# Autodesk Inventor assembly: blocoRolamentoLinearCarroMesa
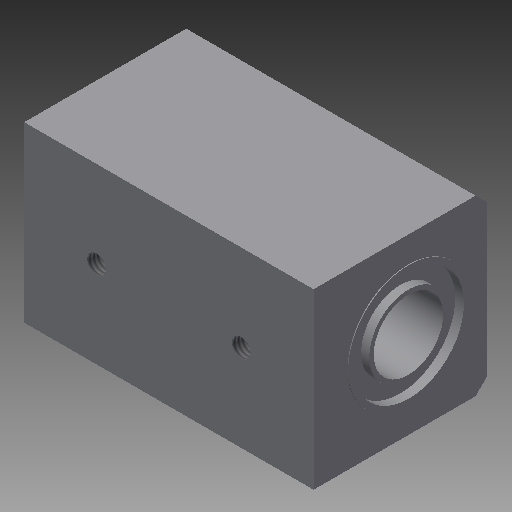
[picture p0: Inventor's stored thumbnail of the model, 512x512]
Saved by Autodesk Inventor 2018 (Build 220112000, 112)
## iProperties
Created: 2018-08-27
Part Number: blocoRolamentoLinearCarroMesa
Material: Genérico
Document SubType Name: Assembly
Designer: Georgines
Author: Georgines
## Documents named in this file (4)
- C:\Users\Georgines\Documents\EstacaoBGA\Peças 3D\blocoRolamentoLinearCarroMesa.iam
- C:\Users\Georgines\Documents\EstacaoBGA\Peças 3D\blocoSuporteRolamentos.ipt
- C:\Users\Georgines\Documents\EstacaoBGA\Peças 3D\rolamento_linear_lm12uu.iam.ipt
- rolamento_linear_lm12uu.iam
## Components (2 placed, 2 different names)
1. blocoSuporteRolamentos:1 — Inserir:1
2. rolamento_linear_lm12uu.iam:1 — Inserir:1
## Relationships (1: Insert 1)
- Inserir:1: blocoSuporteRolamentos:1 ↔ rolamento_linear_lm12uu.iam:1
